# Autodesk Inventor assembly: złożenie gaz
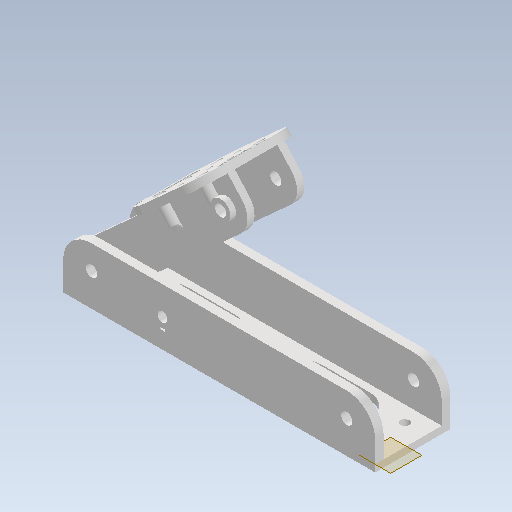
[picture p0: Inventor's stored thumbnail of the model, 512x512]
Saved by Autodesk Inventor 2021 (Build 250183000, 183)
## iProperties
Created: 2022-04-14
Part Number: złożenie gaz
Document SubType Name: Assembly
Designer: Łukasz
Author: Łukasz
## Documents named in this file (5)
- E:\Pliki inventor i stl\motion platform\złożenie gaz.iam
- E:\Pliki inventor i stl\pliki inventor\Kierownica\pedały\baza.ipt
- E:\Pliki inventor i stl\pliki inventor\Kierownica\pedały\pedał nakładka.ipt
- E:\Pliki inventor i stl\pliki inventor\Kierownica\pedały\pedał ruchomy lewy.ipt
- E:\Pliki inventor i stl\pliki inventor\Kierownica\pedały\pedał ruchomy prawy.ipt
## Components (4 placed, 4 different names)
1. baza:1 — Rotational:5
2. pedał nakładka:1 — Rotational:1, Rotational:2, Rotational:3, Rotational:4
3. pedał ruchomy lewy:1 — Rotational:1, Rotational:2
4. pedał ruchomy prawy:1 — Rotational:3, Rotational:4, Rotational:5
## Relationships (5: RevoluteJoint 5)
- Rotational:1 [RevoluteJoint]: pedał nakładka:1 ↔ pedał ruchomy lewy:1
- Rotational:2 [RevoluteJoint]: pedał nakładka:1 ↔ pedał ruchomy lewy:1
- Rotational:3 [RevoluteJoint]: pedał nakładka:1 ↔ pedał ruchomy prawy:1
- Rotational:4 [RevoluteJoint]: pedał nakładka:1 ↔ pedał ruchomy prawy:1
- Rotational:5 [RevoluteJoint]: baza:1 ↔ pedał ruchomy prawy:1
